# Autodesk Inventor assembly: ALU
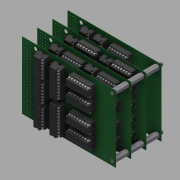
[picture p0: Inventor's stored thumbnail of the model, 180x180]
Saved by Autodesk Inventor 2019.4 (Build 234330000, 330)
## iProperties
Created: 2021-09-13
Part Number: ALU
Document SubType Name: Assembly
Designer: erics
Mass: 51.9566 g
Surface Area: 1600.04 cm^2
Volume: 51.9566 cm^3
Density: 1 g/cm^3
Author: erics
## Documents named in this file (6)
- D:\Users\erics\Documents\16B\Mechanical\ALU.iam
- D:\Users\erics\Documents\16B\ALU_Adder_ZF\ALU_Adder_ZF.iam
- D:\Users\erics\Documents\16B\ALU_AND_OR\ALU_AND_OR.iam
- D:\Users\erics\Documents\16B\ALU_Shifter\ALU_Shifter.iam
- D:\Users\erics\Documents\16B\ALU_XOR_ONES\ALU_XOR_ONES.iam
- D:\Users\erics\Documents\16B\Mechanical\93655A013_Male-Female Threaded Hex Standoff.ipt
## Components (10 placed, 5 different names)
1. ALU_Adder_ZF:1 [sub-assembly] — Mate:1, Mate:2, Mate:5, Mate:6
2. ALU_AND_OR:1 [sub-assembly] — Mate:1, Mate:2, Mate:3, Mate:5, Mate:6, Mate:7, Mate:8, Insert:2, Insert:5
3. ALU_Shifter:1 [sub-assembly] — Mate:3, Mate:4, Mate:7, Mate:8, Mate:9, Mate:10, Insert:1, Insert:4
4. ALU_XOR_ONES:1 [sub-assembly] — Mate:4, Mate:9, Mate:10, Mate:11, Mate:12, Insert:3
5. 93655A013_Male-Female Threaded Hex Standoff:1 — Mate:11, Mate:12
6. 93655A013_Male-Female Threaded Hex Standoff:2 — Insert:1
7. 93655A013_Male-Female Threaded Hex Standoff:3 — Insert:2
8. 93655A013_Male-Female Threaded Hex Standoff:4 — Insert:3
9. 93655A013_Male-Female Threaded Hex Standoff:5 — Insert:4
10. 93655A013_Male-Female Threaded Hex Standoff:6 — Insert:5
## Relationships (17: Mate 12, Insert 5)
- Mate:1: ALU_Adder_ZF:1 ↔ ALU_AND_OR:1
- Mate:2: ALU_Adder_ZF:1 ↔ ALU_AND_OR:1
- Mate:3: ALU_AND_OR:1 ↔ ALU_Shifter:1
- Mate:4: ALU_Shifter:1 ↔ ALU_XOR_ONES:1
- Mate:5: ALU_Adder_ZF:1 ↔ ALU_AND_OR:1
- Mate:6: ALU_Adder_ZF:1 ↔ ALU_AND_OR:1
- Mate:7: ALU_AND_OR:1 ↔ ALU_Shifter:1
- Mate:8: ALU_AND_OR:1 ↔ ALU_Shifter:1
- Mate:9: ALU_Shifter:1 ↔ ALU_XOR_ONES:1
- Mate:10: ALU_Shifter:1 ↔ ALU_XOR_ONES:1
- Mate:11: ALU_XOR_ONES:1 ↔ 93655A013_Male-Female Threaded Hex Standoff:1
- Mate:12: ALU_XOR_ONES:1 ↔ 93655A013_Male-Female Threaded Hex Standoff:1
- Insert:1: ALU_Shifter:1 ↔ 93655A013_Male-Female Threaded Hex Standoff:2
- Insert:2: ALU_AND_OR:1 ↔ 93655A013_Male-Female Threaded Hex Standoff:3
- Insert:3: ALU_XOR_ONES:1 ↔ 93655A013_Male-Female Threaded Hex Standoff:4
- Insert:4: ALU_Shifter:1 ↔ 93655A013_Male-Female Threaded Hex Standoff:5
- Insert:5: ALU_AND_OR:1 ↔ 93655A013_Male-Female Threaded Hex Standoff:6
## Named parameters: Spacing = 28 mm
